# Autodesk Inventor assembly: Z assembly
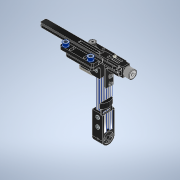
[picture p0: Inventor's stored thumbnail of the model, 180x180]
Saved by Autodesk Inventor 2022 (Build 260153000, 153)
## iProperties
Created: 2022-03-06
Part Number: Z assembly
Document SubType Name: Assembly
Designer: JK
Author: JK
## Documents named in this file (28)
- C:\Users\JK\Documents\Inventor\ScaraNema\SCARA-3DP\Parts\Forearm\Forearm assembly.iam
- C:\Users\JK\Documents\Inventor\ScaraNema\SCARA-3DP\Parts\Forearm\Z Motor support.ipt
- C:\Users\JK\Documents\Inventor\ScaraNema\SCARA-3DP\Parts\V-Slot 20x20.ipt
- C:\Users\JK\Documents\Inventor\ScaraNema\SCARA-3DP\Parts\Forearm\Z axis limit switch support.ipt
- C:\Users\JK\Documents\Inventor\ScaraNema\SCARA-3DP\Parts\Common components\V-Slot 20x20\V-Slot 20x20x150.ipt
- C:\Users\JK\Documents\Inventor\ScaraNema\SCARA-3DP\Parts\Forearm\Forearm support.ipt
- C:\Users\JK\Documents\Inventor\ScaraNema\SCARA-3DP\Parts\Common components\Limit switch.ipt
- C:\Users\JK\Documents\Inventor\ScaraNema\SCARA-3DP\Parts\Fasteners\M2x10 socket bolt.ipt
- C:\Users\JK\Documents\Inventor\ScaraNema\SCARA-3DP\Parts\Fasteners\M2 Hex nut.ipt
- C:\Users\JK\Documents\Inventor\ScaraNema\SCARA-3DP\Parts\Fasteners\M3x10 set screw.ipt
- C:\Users\JK\Documents\Inventor\ScaraNema\SCARA-3DP\Parts\Fasteners\M5x15 Flat head bolt.ipt
- C:\Users\JK\Documents\Inventor\ScaraNema\SCARA-3DP\Parts\Fasteners\M5x10 Flat head bolt.ipt
- C:\Users\JK\Documents\Inventor\ScaraNema\SCARA-3DP\Parts\Fasteners\M5x8 Flat head bolt.ipt
- C:\Users\JK\Documents\Inventor\ScaraNema\SCARA-3DP\Parts\Fasteners\M3 Hex nut.ipt
- C:\Users\JK\Documents\Inventor\ScaraNema\SCARA-3DP\Parts\Fasteners\M5 T-Nut Drop-in 20x20.ipt
- C:\Users\JK\Documents\Inventor\ScaraNema\SCARA-3DP\Parts\Fasteners\M3x6 socket bolt.ipt
- C:\Users\JK\Documents\Inventor\ScaraNema\SCARA-3DP\Parts\Forearm\yystop.ipt
- C:\Users\JK\Documents\Inventor\ScaraNema\SCARA-3DP\Parts\Forearm\Nema14 Stepper Motor v1.ipt
- C:\Users\JK\Documents\Inventor\ScaraNema\SCARA-3DP\Parts\Common components\GT2 16 Pulley.ipt
- C:\Users\JK\Documents\Inventor\ScaraNema\SCARA-3DP\Parts\Forearm\GT2RackA.ipt
- C:\Users\JK\Documents\Inventor\ScaraNema\SCARA-3DP\Parts\Forearm\tococo.ipt
- C:\Users\JK\Documents\Inventor\ScaraNema\SCARA-3DP\Parts\Forearm\GT2RackB.ipt
- C:\Users\JK\Documents\Inventor\ScaraNema\SCARA-3DP\Parts\Forearm\Rack support.ipt
- C:\Users\JK\Documents\Inventor\ScaraNema\SCARA-3DP\Parts\Forearm\magnetsupport.ipt
- C:\Users\JK\Documents\Inventor\ScaraNema\SCARA-3DP\Parts\Common components\Idle pulley 16\GT2-16 Idle pulley.iam
- C:\Users\JK\Documents\Inventor\ScaraNema\SCARA-3DP\Parts\Forearm\m3x35.ipt
- C:\Users\JK\Documents\Inventor\ScaraNema\SCARA-3DP\Parts\Forearm\m3separator.ipt
- C:\Users\JK\Documents\Inventor\ScaraNema\SCARA-3DP\Parts\Forearm\electromagnet.ipt
## Components (52 placed, 26 different names)
1. Z Motor support:1 — Nivelación:1, Coincidencia:32, Coincidencia:48, Ángulo:19, Coincidencia:91, Coincidencia:92, Coincidencia:93, Coincidencia:94, Coincidencia:95, Coincidencia:96, Coincidencia:103, Coincidencia:104, Coincidencia:117, Tangente:2, Coincidencia:118, Coincidencia:129, Nivelación:29, Nivelación:31
2. V-Slot 20x20x150:1 — Nivelación:1, Coincidencia:17, Coincidencia:18, Ángulo:12, Coincidencia:98, Coincidencia:100, Coincidencia:117, Coincidencia:132, Nivelación:30, Nivelación:31
3. Z axis limit switch support:1 — Ángulo:5, Coincidencia:28, Coincidencia:46, Coincidencia:47, Coincidencia:132, Nivelación:29, Nivelación:30, Coincidencia:133, Coincidencia:134, Ángulo:24, Coincidencia:136, Coincidencia:137
4. Forearm support:1 — Coincidencia:17, Coincidencia:18, Coincidencia:33, Coincidencia:34, Coincidencia:35, Coincidencia:36, Coincidencia:37, Coincidencia:38, Coincidencia:42, Ángulo:8, Coincidencia:43, Coincidencia:44, Coincidencia:45, Ángulo:15, Coincidencia:83, Coincidencia:84, Coincidencia:85, Coincidencia:86, Coincidencia:88, Coincidencia:98, Coincidencia:99, Coincidencia:101, Ángulo:21
5. M2x10 socket bolt:1 — Nivelación:9, Coincidencia:26, Coincidencia:134
6. M2x10 socket bolt:2 — Nivelación:9, Coincidencia:27, Coincidencia:133, Coincidencia:138
7. M2 Hex nut:1 — Coincidencia:27, Nivelación:10, Ángulo:4, Ángulo:5
8. M2 Hex nut:2 — Coincidencia:26, Nivelación:10, Ángulo:4, Coincidencia:28
9. M5x15 Flat head bolt:1 — Coincidencia:32, Coincidencia:73, Coincidencia:93
10. M5x10 Flat head bolt:1 — Coincidencia:33, Nivelación:12, Coincidencia:82, Coincidencia:86
11. M5x10 Flat head bolt:2 — Coincidencia:34, Nivelación:12, Coincidencia:81
12. M5x10 Flat head bolt:3 — Coincidencia:35, Nivelación:11, Coincidencia:77, Coincidencia:88
13. M5x10 Flat head bolt:4 — Coincidencia:36, Nivelación:11, Coincidencia:78
14. M5x8 Flat head bolt:1 — Coincidencia:37, Nivelación:13, Coincidencia:79, Coincidencia:99
15. M5x8 Flat head bolt:2 — Coincidencia:38, Nivelación:13, Coincidencia:80
16. M5x8 Flat head bolt:3 — Coincidencia:47, Nivelación:15, Coincidencia:75
17. M5x8 Flat head bolt:4 — Coincidencia:46, Nivelación:15, Coincidencia:74
18. M5x15 Flat head bolt:2 — Coincidencia:48, Coincidencia:76, Coincidencia:94
19. M5 T-Nut Drop-in 20x20:1 — Coincidencia:73, Coincidencia:91
20. M5 T-Nut Drop-in 20x20:2 — Coincidencia:74, Nivelación:22, Ángulo:18, Ángulo:19
21. M5 T-Nut Drop-in 20x20:3 — Coincidencia:75, Nivelación:22, Ángulo:18
22. M5 T-Nut Drop-in 20x20:4 — Coincidencia:76, Coincidencia:92
23. M5 T-Nut Drop-in 20x20:5 — Coincidencia:77, Ángulo:13, Nivelación:25, Ángulo:14, Ángulo:17, Coincidencia:84
24. M5 T-Nut Drop-in 20x20:6 — Coincidencia:78, Ángulo:13, Nivelación:25, Ángulo:14, Ángulo:15
25. M5 T-Nut Drop-in 20x20:7 — Coincidencia:79, Nivelación:23, Ángulo:11, Coincidencia:85
26. M5 T-Nut Drop-in 20x20:8 — Coincidencia:80, Nivelación:23, Ángulo:11, Ángulo:12
27. M5 T-Nut Drop-in 20x20:9 — Coincidencia:82, Nivelación:24, Ángulo:16, Coincidencia:83
28. M5 T-Nut Drop-in 20x20:10 — Coincidencia:81, Nivelación:24, Ángulo:16, Ángulo:17
29. yystop:1 — Coincidencia:100, Coincidencia:101
30. Nema14 Stepper Motor v1:1 — Coincidencia:103, Coincidencia:104, Coincidencia:105, Nivelación:26
31. GT2 16 Pulley:1 — Coincidencia:105, Nivelación:26, Tangente:1, Coincidencia:116
32. GT2RackA:1 — Coincidencia:106, Ángulo:20, Coincidencia:107, Nivelación:27, Coincidencia:108, Coincidencia:109, Tangente:1, Coincidencia:116, Ángulo:22
33. tococo:1 — Nivelación:27, Coincidencia:108, Coincidencia:109
34. GT2RackB:1 — Coincidencia:106, Ángulo:20, Coincidencia:107, Coincidencia:126, Ángulo:23, Coincidencia:130, Coincidencia:139
35. Rack support:1 — Tangente:2, Coincidencia:118, Ángulo:21, Ángulo:22, Coincidencia:127, Coincidencia:128, Coincidencia:129, Coincidencia:131
36. magnetsupport:1 — Coincidencia:126, Ángulo:23, Coincidencia:130, Coincidencia:140, Coincidencia:142, Coincidencia:143, Coincidencia:144
37. GT2-16 Idle pulley:1 [sub-assembly] — Coincidencia:127, Nivelación:28, Coincidencia:131
38. GT2-16 Idle pulley:2 [sub-assembly] — Coincidencia:128, Nivelación:28
39. Limit switch:2 — Ángulo:24, Coincidencia:136, Coincidencia:137, Coincidencia:138
40. m3x35:1 — Coincidencia:139, Coincidencia:140, Coincidencia:141
41. m3separator:1 — Coincidencia:141, Coincidencia:142
42. electromagnet:1 — Coincidencia:143, Coincidencia:144
43. M3x10 set screw:5 — Coincidencia:44, Coincidencia:45
44. M3 Hex nut:1 — Coincidencia:42, Ángulo:8, Coincidencia:43
45. M3x10 set screw:6
46. M3 Hex nut:4
47. M3x10 set screw:7
48. M3 Hex nut:5
49. M3x6 socket bolt:2 — Coincidencia:95, Coincidencia:96
50. M3x6 socket bolt:3
51. M3x6 socket bolt:4
52. M3x6 socket bolt:5
## Component patterns: (3 elements, first: M3x10 set screw:5 + M3 Hex nut:1), (4 elements, first: M3x6 socket bolt:2)
## Relationships (108: Mate 72, Flush 17, Angle 17, Tangent 2)
- Nivelación:1 [Flush]: Z Motor support:1 ↔ V-Slot 20x20x150:1
- Coincidencia:17 [Mate]: V-Slot 20x20x150:1 ↔ Forearm support:1
- Coincidencia:18 [Mate] (0.15 mm): V-Slot 20x20x150:1 ↔ Forearm support:1
- Nivelación:9 [Flush]: M2x10 socket bolt:1 ↔ M2x10 socket bolt:2
- Coincidencia:26 [Mate]: M2x10 socket bolt:1 ↔ M2 Hex nut:2
- Coincidencia:27 [Mate]: M2x10 socket bolt:2 ↔ M2 Hex nut:1
- Nivelación:10 [Flush]: M2 Hex nut:1 ↔ M2 Hex nut:2
- Ángulo:4 [Angle] (0 deg): M2 Hex nut:1 ↔ M2 Hex nut:2
- Ángulo:5 [Angle] (0 deg): Z axis limit switch support:1 ↔ M2 Hex nut:1
- Coincidencia:28 [Mate]: Z axis limit switch support:1 ↔ M2 Hex nut:2
- Coincidencia:32 [Mate]: Z Motor support:1 ↔ M5x15 Flat head bolt:1
- Coincidencia:33 [Mate]: Forearm support:1 ↔ M5x10 Flat head bolt:1
- Coincidencia:34 [Mate]: Forearm support:1 ↔ M5x10 Flat head bolt:2
- Coincidencia:35 [Mate]: Forearm support:1 ↔ M5x10 Flat head bolt:3
- Coincidencia:36 [Mate]: Forearm support:1 ↔ M5x10 Flat head bolt:4
- Nivelación:11 [Flush]: M5x10 Flat head bolt:3 ↔ M5x10 Flat head bolt:4
- Nivelación:12 [Flush]: M5x10 Flat head bolt:1 ↔ M5x10 Flat head bolt:2
- Coincidencia:37 [Mate]: Forearm support:1 ↔ M5x8 Flat head bolt:1
- Coincidencia:38 [Mate]: Forearm support:1 ↔ M5x8 Flat head bolt:2
- Nivelación:13 [Flush]: M5x8 Flat head bolt:1 ↔ M5x8 Flat head bolt:2
- Coincidencia:42 [Mate]: Forearm support:1 ↔ M3 Hex nut:1
- Ángulo:8 [Angle] (0 deg): Forearm support:1 ↔ M3 Hex nut:1
- Coincidencia:43 [Mate]: Forearm support:1 ↔ M3 Hex nut:1
- Coincidencia:44 [Mate]: Forearm support:1 ↔ M3x10 set screw:5
- Coincidencia:45 [Mate] (-5 mm): Forearm support:1 ↔ M3x10 set screw:5
- Coincidencia:46 [Mate]: Z axis limit switch support:1 ↔ M5x8 Flat head bolt:4
- Coincidencia:47 [Mate]: Z axis limit switch support:1 ↔ M5x8 Flat head bolt:3
- Nivelación:15 [Flush]: M5x8 Flat head bolt:3 ↔ M5x8 Flat head bolt:4
- Coincidencia:48 [Mate]: Z Motor support:1 ↔ M5x15 Flat head bolt:2
- Coincidencia:73 [Mate]: M5x15 Flat head bolt:1 ↔ M5 T-Nut Drop-in 20x20:1
- Coincidencia:74 [Mate]: M5x8 Flat head bolt:4 ↔ M5 T-Nut Drop-in 20x20:2
- Coincidencia:75 [Mate]: M5x8 Flat head bolt:3 ↔ M5 T-Nut Drop-in 20x20:3
- Coincidencia:76 [Mate]: M5x15 Flat head bolt:2 ↔ M5 T-Nut Drop-in 20x20:4
- Nivelación:22 [Flush]: M5 T-Nut Drop-in 20x20:2 ↔ M5 T-Nut Drop-in 20x20:3
- Coincidencia:77 [Mate]: M5x10 Flat head bolt:3 ↔ M5 T-Nut Drop-in 20x20:5
- Coincidencia:78 [Mate]: M5x10 Flat head bolt:4 ↔ M5 T-Nut Drop-in 20x20:6
- Coincidencia:79 [Mate]: M5x8 Flat head bolt:1 ↔ M5 T-Nut Drop-in 20x20:7
- Coincidencia:80 [Mate]: M5x8 Flat head bolt:2 ↔ M5 T-Nut Drop-in 20x20:8
- Coincidencia:81 [Mate]: M5x10 Flat head bolt:2 ↔ M5 T-Nut Drop-in 20x20:10
- Coincidencia:82 [Mate]: M5x10 Flat head bolt:1 ↔ M5 T-Nut Drop-in 20x20:9
- Nivelación:23 [Flush]: M5 T-Nut Drop-in 20x20:7 ↔ M5 T-Nut Drop-in 20x20:8
- Nivelación:24 [Flush]: M5 T-Nut Drop-in 20x20:9 ↔ M5 T-Nut Drop-in 20x20:10
- Ángulo:11 [Angle] (0 deg): M5 T-Nut Drop-in 20x20:7 ↔ M5 T-Nut Drop-in 20x20:8
- Ángulo:12 [Angle] (90 deg): V-Slot 20x20x150:1 ↔ M5 T-Nut Drop-in 20x20:8
- Ángulo:13 [Angle] (0 deg): M5 T-Nut Drop-in 20x20:5 ↔ M5 T-Nut Drop-in 20x20:6
- Nivelación:25 [Flush]: M5 T-Nut Drop-in 20x20:5 ↔ M5 T-Nut Drop-in 20x20:6
- Ángulo:14 [Angle] (0 deg): M5 T-Nut Drop-in 20x20:5 ↔ M5 T-Nut Drop-in 20x20:6
- Ángulo:15 [Angle] (0 deg): Forearm support:1 ↔ M5 T-Nut Drop-in 20x20:6
- Ángulo:16 [Angle] (0 deg): M5 T-Nut Drop-in 20x20:9 ↔ M5 T-Nut Drop-in 20x20:10
- Ángulo:17 [Angle] (0 deg): M5 T-Nut Drop-in 20x20:5 ↔ M5 T-Nut Drop-in 20x20:10
- Coincidencia:83 [Mate] (0.6 mm): Forearm support:1 ↔ M5 T-Nut Drop-in 20x20:9
- Coincidencia:84 [Mate] (0.6 mm): Forearm support:1 ↔ M5 T-Nut Drop-in 20x20:5
- Coincidencia:85 [Mate] (0.6 mm): Forearm support:1 ↔ M5 T-Nut Drop-in 20x20:7
- Coincidencia:86 [Mate]: Forearm support:1 ↔ M5x10 Flat head bolt:1
- Coincidencia:88 [Mate]: Forearm support:1 ↔ M5x10 Flat head bolt:3
- Ángulo:18 [Angle] (0 deg): M5 T-Nut Drop-in 20x20:2 ↔ M5 T-Nut Drop-in 20x20:3
- Ángulo:19 [Angle] (0 deg): Z Motor support:1 ↔ M5 T-Nut Drop-in 20x20:2
- Coincidencia:91 [Mate] (0.6 mm): Z Motor support:1 ↔ M5 T-Nut Drop-in 20x20:1
- Coincidencia:92 [Mate] (0.6 mm): Z Motor support:1 ↔ M5 T-Nut Drop-in 20x20:4
- Coincidencia:93 [Mate]: Z Motor support:1 ↔ M5x15 Flat head bolt:1
- Coincidencia:94 [Mate]: Z Motor support:1 ↔ M5x15 Flat head bolt:2
- Coincidencia:95 [Mate]: Z Motor support:1 ↔ M3x6 socket bolt:2
- Coincidencia:96 [Mate]: Z Motor support:1 ↔ M3x6 socket bolt:2
- Coincidencia:98 [Mate]: V-Slot 20x20x150:1 ↔ Forearm support:1
- Coincidencia:99 [Mate]: Forearm support:1 ↔ M5x8 Flat head bolt:1
- Coincidencia:100 [Mate] (5 mm): V-Slot 20x20x150:1 ↔ yystop:1
- Coincidencia:101 [Mate] (20 mm): Forearm support:1 ↔ yystop:1
- Coincidencia:103 [Mate]: Z Motor support:1 ↔ Nema14 Stepper Motor v1:1
- Coincidencia:104 [Mate]: Z Motor support:1 ↔ Nema14 Stepper Motor v1:1
- Coincidencia:105 [Mate]: Nema14 Stepper Motor v1:1 ↔ GT2 16 Pulley:1
- Nivelación:26 [Flush]: Nema14 Stepper Motor v1:1 ↔ GT2 16 Pulley:1
- Coincidencia:106 [Mate]: GT2RackA:1 ↔ GT2RackB:1
- Ángulo:20 [Angle] (0 deg): GT2RackA:1 ↔ GT2RackB:1
- Coincidencia:107 [Mate] (1 mm): GT2RackA:1 ↔ GT2RackB:1
- Nivelación:27 [Flush]: GT2RackA:1 ↔ tococo:1
- Coincidencia:108 [Mate]: GT2RackA:1 ↔ tococo:1
- Coincidencia:109 [Mate] (0.15 mm): GT2RackA:1 ↔ tococo:1
- Tangente:1 (-0.5 mm): GT2 16 Pulley:1 ↔ GT2RackA:1
- Coincidencia:116 [Mate] (0.5 mm): GT2 16 Pulley:1 ↔ GT2RackA:1
- Coincidencia:117 [Mate] (0.15 mm): Z Motor support:1 ↔ V-Slot 20x20x150:1
- Tangente:2: Z Motor support:1 ↔ Rack support:1
- Coincidencia:118 [Mate]: Z Motor support:1 ↔ Rack support:1
- Ángulo:21 [Angle] (0 deg): Forearm support:1 ↔ Rack support:1
- Ángulo:22 [Angle] (0 deg): GT2RackA:1 ↔ Rack support:1
- Coincidencia:126 [Mate] (0.15 mm): GT2RackB:1 ↔ magnetsupport:1
- Ángulo:23 [Angle] (0 deg): GT2RackB:1 ↔ magnetsupport:1
- Coincidencia:127 [Mate]: Rack support:1 ↔ GT2-16 Idle pulley:1
- Coincidencia:128 [Mate]: Rack support:1 ↔ GT2-16 Idle pulley:2
- Nivelación:28 [Flush]: GT2-16 Idle pulley:1 ↔ GT2-16 Idle pulley:2
- Coincidencia:129 [Mate]: Z Motor support:1 ↔ Rack support:1
- Coincidencia:130 [Mate]: GT2RackB:1 ↔ magnetsupport:1
- Coincidencia:131 [Mate] (1.2 mm): Rack support:1 ↔ GT2-16 Idle pulley:1
- Coincidencia:132 [Mate]: V-Slot 20x20x150:1 ↔ Z axis limit switch support:1
- Nivelación:29 [Flush] (7 mm): Z Motor support:1 ↔ Z axis limit switch support:1
- Nivelación:30 [Flush]: V-Slot 20x20x150:1 ↔ Z axis limit switch support:1
- Nivelación:31 [Flush]: Z Motor support:1 ↔ V-Slot 20x20x150:1
- Coincidencia:133 [Mate]: Z axis limit switch support:1 ↔ M2x10 socket bolt:2
- Coincidencia:134 [Mate]: Z axis limit switch support:1 ↔ M2x10 socket bolt:1
- Ángulo:24 [Angle] (0 deg): Z axis limit switch support:1 ↔ Limit switch:2
- Coincidencia:136 [Mate]: Z axis limit switch support:1 ↔ Limit switch:2
- Coincidencia:137 [Mate]: Z axis limit switch support:1 ↔ Limit switch:2
- Coincidencia:138 [Mate]: M2x10 socket bolt:2 ↔ Limit switch:2
- Coincidencia:139 [Mate]: GT2RackB:1 ↔ m3x35:1
- Coincidencia:140 [Mate]: magnetsupport:1 ↔ m3x35:1
- Coincidencia:141 [Mate]: m3x35:1 ↔ m3separator:1
- Coincidencia:142 [Mate]: magnetsupport:1 ↔ m3separator:1
- Coincidencia:143 [Mate]: magnetsupport:1 ↔ electromagnet:1
- Coincidencia:144 [Mate]: magnetsupport:1 ↔ electromagnet:1
